# Autodesk Inventor assembly: motor
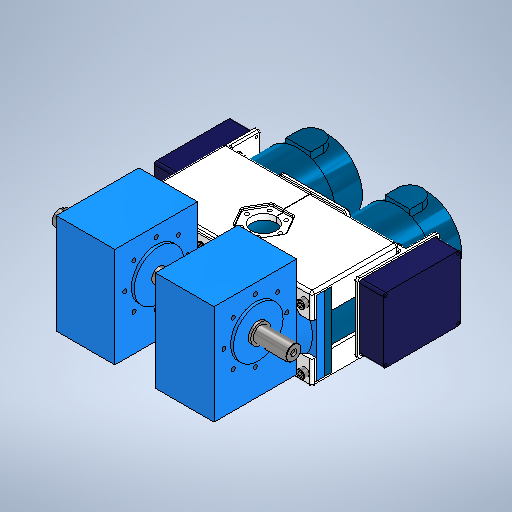
[picture p0: Inventor's stored thumbnail of the model, 512x512]
Saved by Autodesk Inventor 2025.3 (Build 293356030, 356C)
## iProperties
Created: 2025-09-06
Part Number: motor
Document SubType Name: Assembly
Designer: MSI
Mass: 13635.5 g
Surface Area: 5600.72 cm^2
Volume: 4817.73 cm^3
Density: 2.83028 g/cm^3
Author: MSI
## Documents named in this file (13)
- C:\Users\MSI\Desktop\Project\3. 로봇팔\Robot Arm Model\joint3\motor.iam
- C:\Users\MSI\Desktop\Project\3. 로봇팔\Robot Arm Model\joint4\NMRV30_motor.iam
- C:\Users\MSI\Desktop\Project\3. 로봇팔\Robot Arm Model\joint4\motor_shaft.ipt
- C:\Users\MSI\Desktop\Project\3. 로봇팔\Robot Arm Model\joint4\motor_driver.ipt
- C:\Users\MSI\Documents\Inventor\Content Center Files\R2025\ko-KR\ISO 4762(2)\ISO 4762 - M6 x 30ISO.ipt
- C:\Users\MSI\Documents\Inventor\Content Center Files\R2025\ko-KR\ISO 4032(2)\ISO 4032 - M6 - ISO.ipt
- C:\Users\MSI\Desktop\Project\3. 로봇팔\Robot Arm Model\joint3\motor_driver_frame.ipt
- C:\Users\MSI\Desktop\Project\3. 로봇팔\Robot Arm Model\joint3\motor_clamp1.ipt
- C:\Users\MSI\Desktop\Project\3. 로봇팔\Robot Arm Model\joint3\motor_clamp2.ipt
- C:\Users\MSI\Documents\Inventor\Content Center Files\R2025\ko-KR\ISO 7045  H\ISO 7045 - M4 x 25_ - 4.8 - H - ISO.ipt
- C:\Users\MSI\Desktop\Project\3. 로봇팔\Robot Arm Model\joint3\motor_holder1.ipt
- C:\Users\MSI\Desktop\Project\3. 로봇팔\Robot Arm Model\joint3\motor_holder2.ipt
- C:\Users\MSI\Desktop\Project\3. 로봇팔\Robot Arm Model\joint3\carbon.ipt
## Components (42 placed, 12 different names)
1. NMRV30_motor:1 [sub-assembly] — 회전:2, 메이트:2, 삽입:27, 삽입:30
2. NMRV30_motor:2 [sub-assembly] — 회전:1, 메이트:1, 삽입:28, 삽입:29
3. motor_holder1:1 — 메이트:5, 메이트:6, 플러쉬:1, 메이트:8, 각도:3, 삽입:8, 삽입:7, 삽입:17, 삽입:28
4. motor_holder2:1 — 플러쉬:1, 메이트:7, 메이트:8, 삽입:5, 삽입:6, 각도:4, 삽입:13, 삽입:23, 삽입:27
5. motor_holder1:2 — 메이트:10, 메이트:11, 삽입:1, 각도:2, 메이트:4, 삽입:2, 삽입:14, 삽입:30
6. motor_holder2:2 — 삽입:3, 삽입:4, 각도:1, 메이트:12, 메이트:13, 삽입:18, 삽입:24, 삽입:29
7. motor_shaft:1 — 회전:1
8. motor_shaft:2 — 회전:2
9. motor_driver:1 — 삽입:19, 삽입:20
10. motor_driver:2 — 삽입:15, 삽입:16
11. motor_driver_frame:1 — 삽입:13, 삽입:14, 삽입:15, 삽입:16, 삽입:25
12. motor_driver_frame:2 — 삽입:17, 삽입:18, 삽입:19, 삽입:20
13. motor_clamp1:1 — 삽입:21, 삽입:22
14. motor_clamp2:1 — 삽입:23, 삽입:24, 삽입:26
15. ISO 4762 M6 x 30:1 — 삽입:4
16. ISO 4762 M6 x 30:2 — 삽입:5
17. ISO 4762 M6 x 30:3 — 삽입:3, 삽입:9
18. ISO 4762 M6 x 30:4 — 삽입:6, 삽입:12
19. ISO 4762 M6 x 30:5 — 삽입:8
20. ISO 4762 M6 x 30:6 — 삽입:1
21. ISO 4762 M6 x 30:7 — 삽입:7, 삽입:11, 삽입:21
22. ISO 4762 M6 x 30:8 — 삽입:2, 삽입:10, 삽입:22
23. ISO 4032 M6:1 — 삽입:12, 각도:4
24. ISO 4032 M6:2 — 삽입:9, 각도:1
25. ISO 4032 M6:3 — 삽입:11, 각도:3
26. ISO 4032 M6:4 — 삽입:10, 각도:2
27. ISO 7045 H M4 x 25 - 4.8 - H:5
28. ISO 7045 H M4 x 25 - 4.8 - H:6
29. ISO 7045 H M4 x 25 - 4.8 - H:7
30. ISO 7045 H M4 x 25 - 4.8 - H:8
31. carbon:1 — 메이트:5, 메이트:6, 메이트:7
32. carbon:2
33. carbon:3
34. carbon:4
35. carbon:5 — 메이트:10, 메이트:11, 메이트:12
36. carbon:6
37. carbon:7
38. carbon:8
39. ISO 7045 H M4 x 25 - 4.8 - H:2 — 삽입:26
40. ISO 7045 H M4 x 25 - 4.8 - H:1 — 삽입:25
41. ISO 7045 H M4 x 25 - 4.8 - H:3
42. ISO 7045 H M4 x 25 - 4.8 - H:4
## Component patterns: (4 elements, first: carbon:1), (4 elements, first: carbon:5), (2 elements, first: ISO 7045 H M4 x 25 - 4.8 - H:2 + ISO 7045 H M4 x 25 - 4.8 - H:1)
## Relationships (50: Insert 30, Mate 12, Angle 4, RevoluteJoint 2, Flush 2)
- 회전:1 [RevoluteJoint]: NMRV30_motor:2 ↔ motor_shaft:1
- 회전:2 [RevoluteJoint]: NMRV30_motor:1 ↔ motor_shaft:2
- 메이트:1 [Mate]: NMRV30_motor:2
- 삽입:1 [Insert]: motor_holder1:2 ↔ ISO 4762 M6 x 30:6
- 삽입:2 [Insert]: motor_holder1:2 ↔ ISO 4762 M6 x 30:8
- 삽입:3 [Insert]: motor_holder2:2 ↔ ISO 4762 M6 x 30:3
- 삽입:4 [Insert]: motor_holder2:2 ↔ ISO 4762 M6 x 30:1
- 삽입:5 [Insert]: motor_holder2:1 ↔ ISO 4762 M6 x 30:2
- 삽입:6 [Insert]: motor_holder2:1 ↔ ISO 4762 M6 x 30:4
- 삽입:7 [Insert]: motor_holder1:1 ↔ ISO 4762 M6 x 30:7
- 삽입:8 [Insert]: motor_holder1:1 ↔ ISO 4762 M6 x 30:5
- 삽입:9 [Insert] (-6.5 mm): ISO 4762 M6 x 30:3 ↔ ISO 4032 M6:2
- 각도:1 [Angle] (0 deg): motor_holder2:2 ↔ ISO 4032 M6:2
- 삽입:10 [Insert] (-6.5 mm): ISO 4762 M6 x 30:8 ↔ ISO 4032 M6:4
- 각도:2 [Angle] (0 deg): motor_holder1:2 ↔ ISO 4032 M6:4
- 삽입:11 [Insert] (-6.5 mm): ISO 4762 M6 x 30:7 ↔ ISO 4032 M6:3
- 각도:3 [Angle] (0 deg): motor_holder1:1 ↔ ISO 4032 M6:3
- 삽입:12 [Insert] (-6.5 mm): ISO 4762 M6 x 30:4 ↔ ISO 4032 M6:1
- 각도:4 [Angle] (0 deg): motor_holder2:1 ↔ ISO 4032 M6:1
- 메이트:2 [Mate]: NMRV30_motor:1
- 메이트:13 [Mate]: motor_holder2:2
- 메이트:4 [Mate]: motor_holder1:2
- 삽입:13 [Insert]: motor_holder2:1 ↔ motor_driver_frame:1
- 삽입:14 [Insert]: motor_holder1:2 ↔ motor_driver_frame:1
- 삽입:15 [Insert]: motor_driver:2 ↔ motor_driver_frame:1
- 삽입:16 [Insert]: motor_driver:2 ↔ motor_driver_frame:1
- 삽입:17 [Insert]: motor_holder1:1 ↔ motor_driver_frame:2
- 삽입:18 [Insert]: motor_holder2:2 ↔ motor_driver_frame:2
- 삽입:19 [Insert]: motor_driver:1 ↔ motor_driver_frame:2
- 삽입:20 [Insert]: motor_driver:1 ↔ motor_driver_frame:2
- 삽입:21 [Insert]: motor_clamp1:1 ↔ ISO 4762 M6 x 30:7
- 삽입:22 [Insert]: motor_clamp1:1 ↔ ISO 4762 M6 x 30:8
- 삽입:23 [Insert]: motor_holder2:1 ↔ motor_clamp2:1
- 삽입:24 [Insert]: motor_holder2:2 ↔ motor_clamp2:1
- 삽입:25 [Insert]: motor_driver_frame:1 ↔ ISO 7045 H M4 x 25 - 4.8 - H:1
- 삽입:26 [Insert]: motor_clamp2:1 ↔ ISO 7045 H M4 x 25 - 4.8 - H:2
- 메이트:5 [Mate]: motor_holder1:1 ↔ carbon:1
- 메이트:6 [Mate]: motor_holder1:1 ↔ carbon:1
- 플러쉬:1 [Flush]: motor_holder1:1 ↔ motor_holder2:1
- 메이트:7 [Mate]: motor_holder2:1 ↔ carbon:1
- 메이트:8 [Mate]: motor_holder1:1 ↔ motor_holder2:1
- 삽입:27 [Insert]: NMRV30_motor:1 ↔ motor_holder2:1
- 삽입:28 [Insert]: NMRV30_motor:2 ↔ motor_holder1:1
- [Flush]: motor_holder1:2 ↔ motor_holder2:2
- [Mate]: motor_holder1:2 ↔ motor_holder2:2
- 메이트:10 [Mate]: motor_holder1:2 ↔ carbon:5
- 메이트:11 [Mate]: motor_holder1:2 ↔ carbon:5
- 메이트:12 [Mate]: motor_holder2:2 ↔ carbon:5
- 삽입:29 [Insert]: NMRV30_motor:2 ↔ motor_holder2:2
- 삽입:30 [Insert]: NMRV30_motor:1 ↔ motor_holder1:2
## Named parameters: d84_d78 = 0 mm, d85_d81 = 0 mm
